# Autodesk Inventor assembly: Dętka
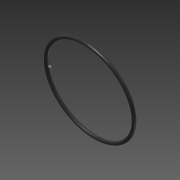
[picture p0: Inventor's stored thumbnail of the model, 180x180]
Saved by Autodesk Inventor 2015 (Build 190159000, 159)
## iProperties
Created: 2015-12-01
Part Number: Dętka
Document SubType Name: Assembly
Designer: graaapsik
Author: graaapsik
## Documents named in this file (3)
- C:\Users\EriveltonDell\Documents\Centro Universitário da FEI\Wheelchair\CADEIRA DE RODAS - DESENHO\Model\Dętka.iam
- C:\Users\EriveltonDell\Documents\Centro Universitário da FEI\Wheelchair\CADEIRA DE RODAS - DESENHO\Model\Dętka_koła_tylnego.ipt
- C:\Users\EriveltonDell\Documents\Centro Universitário da FEI\Wheelchair\CADEIRA DE RODAS - DESENHO\Model\Wentyl.iam
## Components (2 placed, 2 different names)
1. Dętka_koła_tylnego:1 — Walcowe:1, Sztywne:1
2. Wentyl:1 [sub-assembly] — Walcowe:1, Sztywne:1
## Relationships (2: CylindricalJoint 1, WeldJoint 1)
- Walcowe:1 [CylindricalJoint]: Dętka_koła_tylnego:1 ↔ Wentyl:1
- Sztywne:1 [WeldJoint]: Dętka_koła_tylnego:1 ↔ Wentyl:1
